# Autodesk Inventor assembly: head-assembly
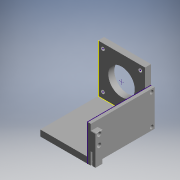
[picture p0: Inventor's stored thumbnail of the model, 180x180]
Saved by Autodesk Inventor 2016 (Build 200138000, 138)
## iProperties
Created: 2015-04-29
Part Number: head-assembly
Document SubType Name: Assembly
Designer: ax
Author: ax
## Documents named in this file (4)
- C:\Users\ax\Documents\Inventor\mintplacer\head-assembly.iam
- C:\Users\ax\Documents\Inventor\mintplacer\head-baseblate.ipt
- C:\Users\ax\Documents\Inventor\mintplacer\head-sideplate.ipt
- C:\Users\ax\Documents\Inventor\mintplacer\GT2 belt clamp.ipt
## Components (3 placed, 3 different names)
1. head-baseblate:1 — Flush:1
2. head-sideplate:1 — Flush:1, Flush:2, Flush:3, Mate:1
3. GT2 belt clamp:1 — Flush:2, Flush:3, Mate:1
## Relationships (4: Flush 3, Mate 1)
- Flush:1: head-baseblate:1 ↔ head-sideplate:1
- Flush:2: head-sideplate:1 ↔ GT2 belt clamp:1
- Flush:3: head-sideplate:1 ↔ GT2 belt clamp:1
- Mate:1: head-sideplate:1 ↔ GT2 belt clamp:1
